# Autodesk Inventor assembly: Climber
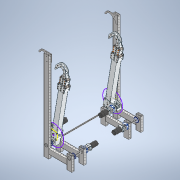
[picture p0: Inventor's stored thumbnail of the model, 180x180]
Saved by Autodesk Inventor 2022 (Build 260153000, 153)
## iProperties
Created: 2022-03-04
Part Number: Climber
Document SubType Name: Assembly
Designer: tagaz
Author: tagaz
## Documents named in this file (11)
- C:\Users\tagaz\OneDrive\Documents\T3-Cad\CAD\2022 Parts\TelescopeElev\Climber.iam
- C:\Users\tagaz\OneDrive\Documents\T3-Cad\CAD\2022 Parts\TelescopeElev\PivotMech\PivotMech.iam
- C:\Users\tagaz\OneDrive\Documents\T3-Cad\CAD\Bearing  for THUNDER.ipt
- C:\Users\tagaz\OneDrive\Documents\T3-Cad\CAD\2022 Parts\TelescopeElev\PivotMech\PivotShaft.ipt
- C:\Users\tagaz\OneDrive\Documents\T3-Cad\CAD\2022 Parts\TelescopeElev\PivotMech\PivotShaft2.ipt
- C:\Users\tagaz\OneDrive\Documents\T3-Cad\CAD\2022 Parts\TelescopeElev\am-4668 2 Stage Climber in a Box2.iam
- C:\Users\tagaz\OneDrive\Documents\T3-Cad\CAD\2022 Parts\TelescopeElev\PivotMech\PivotMech2.iam
- C:\Users\tagaz\OneDrive\Documents\T3-Cad\CAD\2022 Parts\TelescopeElev\FlexiHook.ipt
- C:\Users\tagaz\OneDrive\Documents\T3-Cad\CAD\2022 Parts\TelescopeElev\Hook.ipt
- C:\Users\tagaz\OneDrive\Documents\T3-Cad\CAD\Generic and Stock\VersaPlanetary Parts\VersaPlanetary Two Stage 775.iam
- C:\Users\tagaz\OneDrive\Documents\T3-Cad\CAD\Generic and Stock\15T Sprocket.ipt
## Components (35 placed, 10 different names)
1. PivotMech2:1 [sub-assembly] — Mate:1, Flush:1, Flush:2, Insert:9, Insert:10, Insert:11, Insert:12, Insert:13, Insert:14, Insert:15, Insert:16, Mate:10, Mate:19, Mate:20, Mate:36, Mate:41, Mate:42
2. PivotMech:2 [sub-assembly] — Mate:1, Flush:1, Flush:2, Insert:1, Insert:2, Insert:3, Insert:4, Insert:5, Insert:6, Insert:7, Insert:8, Mate:9, Mate:17, Mate:18, Mate:28, Mate:38, Mate:40
3. Bearing  for THUNDER:1 — Insert:5, Mate:27
4. Bearing  for THUNDER:2 — Insert:4, Flush:7
5. Bearing  for THUNDER:3 — Insert:7
6. Bearing  for THUNDER:4 — Insert:8, Mate:11
7. Bearing  for THUNDER:5 — Insert:1, Mate:3, Flush:5
8. Bearing  for THUNDER:6 — Insert:6, Mate:16
9. Bearing  for THUNDER:7 — Insert:2
10. Bearing  for THUNDER:8 — Insert:3
11. Bearing  for THUNDER:9 — Insert:15
12. Bearing  for THUNDER:10 — Insert:16
13. Bearing  for THUNDER:11 — Insert:14
14. Bearing  for THUNDER:12 — Insert:12, Mate:43
15. Bearing  for THUNDER:13 — Insert:13, Mate:30
16. Bearing  for THUNDER:14 — Insert:10, Mate:12, Mate:44
17. Bearing  for THUNDER:15 — Insert:11, Mate:15
18. Bearing  for THUNDER:16 — Insert:9
19. PivotShaft:2 — Mate:3, Flush:5, Mate:13, Mate:14, Mate:39
20. am-4668 2 Stage Climber in a Box2:1 [sub-assembly] — Mate:10, Mate:12, Mate:13, Mate:21, Mate:25, Mate:26, Mate:31, Mate:34, Mate:35
21. am-4668 2 Stage Climber in a Box2:2 [sub-assembly] — Mate:9, Mate:11, Mate:14, Mate:22, Mate:23, Mate:24, Mate:29, Mate:32, Mate:33
22. PivotShaft2:1 — Mate:15
23. PivotShaft2:2 — Mate:16, Flush:7, Mate:37
24. FlexiHook:1 — Mate:17, Mate:18
25. FlexiHook:2 — Mate:19, Mate:20
26. Hook:1 — Mate:21, Mate:25, Mate:26
27. Hook:2 — Mate:22, Mate:23, Mate:24
28. VersaPlanetary Two Stage 775:1 [sub-assembly] — Mate:27, Mate:28
29. VersaPlanetary Two Stage 775:2 [sub-assembly] — Mate:30, Mate:36
30. VersaPlanetary Two Stage 775:3 [sub-assembly] — Mate:31, Mate:34, Mate:35
31. VersaPlanetary Two Stage 775:4 [sub-assembly] — Mate:29, Mate:32, Mate:33
32. 15T Sprocket:1 — Mate:37, Mate:38
33. 15T Sprocket:2 — Mate:39, Mate:40
34. 15T Sprocket:3 — Mate:42, Mate:43
35. 15T Sprocket:4 — Mate:41, Mate:44
## Relationships (58: Mate 38, Insert 16, Flush 4)
- Mate:1 (444.5 mm): PivotMech2:1 ↔ PivotMech:2
- Flush:1: PivotMech2:1 ↔ PivotMech:2
- Flush:2: PivotMech2:1 ↔ PivotMech:2
- Insert:1: PivotMech:2 ↔ Bearing  for THUNDER:5
- Insert:2: PivotMech:2 ↔ Bearing  for THUNDER:7
- Insert:3: PivotMech:2 ↔ Bearing  for THUNDER:8
- Insert:4: PivotMech:2 ↔ Bearing  for THUNDER:2
- Insert:5: PivotMech:2 ↔ Bearing  for THUNDER:1
- Insert:6: PivotMech:2 ↔ Bearing  for THUNDER:6
- Insert:7: PivotMech:2 ↔ Bearing  for THUNDER:3
- Insert:8: PivotMech:2 ↔ Bearing  for THUNDER:4
- Insert:9: PivotMech2:1 ↔ Bearing  for THUNDER:16
- Insert:10: PivotMech2:1 ↔ Bearing  for THUNDER:14
- Insert:11: PivotMech2:1 ↔ Bearing  for THUNDER:15
- Insert:12: PivotMech2:1 ↔ Bearing  for THUNDER:12
- Insert:13: PivotMech2:1 ↔ Bearing  for THUNDER:13
- Insert:14: PivotMech2:1 ↔ Bearing  for THUNDER:11
- Insert:15: PivotMech2:1 ↔ Bearing  for THUNDER:9
- Insert:16: PivotMech2:1 ↔ Bearing  for THUNDER:10
- Mate:3: Bearing  for THUNDER:5 ↔ PivotShaft:2
- Flush:5: Bearing  for THUNDER:5 ↔ PivotShaft:2
- Mate:9 (44.45 mm): PivotMech:2 ↔ am-4668 2 Stage Climber in a Box2:2
- Mate:10 (44.45 mm): PivotMech2:1 ↔ am-4668 2 Stage Climber in a Box2:1
- Mate:11: Bearing  for THUNDER:4 ↔ am-4668 2 Stage Climber in a Box2:2
- Mate:12: Bearing  for THUNDER:14 ↔ am-4668 2 Stage Climber in a Box2:1
- Mate:13: PivotShaft:2 ↔ am-4668 2 Stage Climber in a Box2:1
- Mate:14: PivotShaft:2 ↔ am-4668 2 Stage Climber in a Box2:2
- Mate:15: Bearing  for THUNDER:15 ↔ PivotShaft2:1
- Mate:16: Bearing  for THUNDER:6 ↔ PivotShaft2:2
- Mate:17: PivotMech:2 ↔ FlexiHook:1
- Mate:18: PivotMech:2 ↔ FlexiHook:1
- Mate:19: PivotMech2:1 ↔ FlexiHook:2
- Mate:20: PivotMech2:1 ↔ FlexiHook:2
- Mate:21: am-4668 2 Stage Climber in a Box2:1 ↔ Hook:1
- Mate:22: am-4668 2 Stage Climber in a Box2:2 ↔ Hook:2
- Mate:23: am-4668 2 Stage Climber in a Box2:2 ↔ Hook:2
- Mate:24: am-4668 2 Stage Climber in a Box2:2 ↔ Hook:2
- Mate:25: am-4668 2 Stage Climber in a Box2:1 ↔ Hook:1
- Mate:26: am-4668 2 Stage Climber in a Box2:1 ↔ Hook:1
- Flush:7: Bearing  for THUNDER:2 ↔ PivotShaft2:2
- Mate:27: Bearing  for THUNDER:1 ↔ VersaPlanetary Two Stage 775:1
- Mate:28: PivotMech:2 ↔ VersaPlanetary Two Stage 775:1
- Mate:29: am-4668 2 Stage Climber in a Box2:2 ↔ VersaPlanetary Two Stage 775:4
- Mate:30: Bearing  for THUNDER:13 ↔ VersaPlanetary Two Stage 775:2
- Mate:31: am-4668 2 Stage Climber in a Box2:1 ↔ VersaPlanetary Two Stage 775:3
- Mate:32: am-4668 2 Stage Climber in a Box2:2 ↔ VersaPlanetary Two Stage 775:4
- Mate:33: am-4668 2 Stage Climber in a Box2:2 ↔ VersaPlanetary Two Stage 775:4
- Mate:34: am-4668 2 Stage Climber in a Box2:1 ↔ VersaPlanetary Two Stage 775:3
- Mate:35: am-4668 2 Stage Climber in a Box2:1 ↔ VersaPlanetary Two Stage 775:3
- Mate:36: PivotMech2:1 ↔ VersaPlanetary Two Stage 775:2
- Mate:37: PivotShaft2:2 ↔ 15T Sprocket:1
- Mate:38 (12.7 mm): PivotMech:2 ↔ 15T Sprocket:1
- Mate:39: PivotShaft:2 ↔ 15T Sprocket:2
- Mate:40 (12.7 mm): PivotMech:2 ↔ 15T Sprocket:2
- Mate:41 (12.7 mm): PivotMech2:1 ↔ 15T Sprocket:4
- Mate:42 (12.7 mm): PivotMech2:1 ↔ 15T Sprocket:3
- Mate:43: Bearing  for THUNDER:12 ↔ 15T Sprocket:3
- Mate:44: Bearing  for THUNDER:14 ↔ 15T Sprocket:4
